# Autodesk Inventor assembly: PIHTI-for-Boron_2026_non-rotating
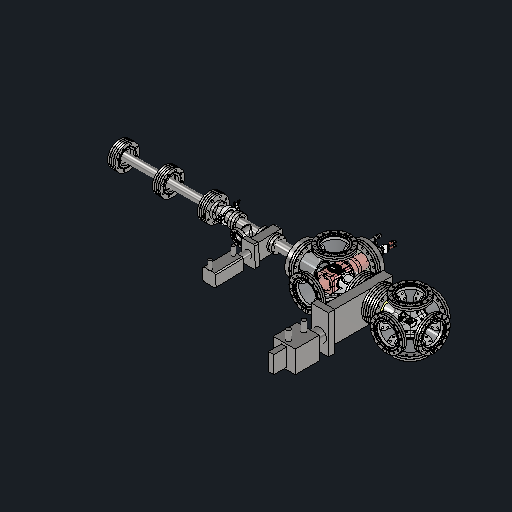
[picture p0: Inventor's stored thumbnail of the model, 512x512]
Saved by Autodesk Inventor 2027.1 (Build 311270010, 270A)
## iProperties
Created: 2024-05-09
Part Number: PIHTI-for-Boron_2026_non-rotating
Document SubType Name: Assembly
Designer: kuzmin
Mass: 19614.5 g
Surface Area: 13609.5 cm^2
Volume: 3689.47 cm^3
Density: 5.31636 g/cm^3
Author: kuzmin
## Documents named in this file (25)
- C:\Users\queezz\Dropbox\Drawings\pihti-cad\Plasma Vessel_2026\PIHTI-for-Boron_2026_non-rotating.iam
- C:\Users\queezz\Dropbox\Drawings\pihti-cad\Plasma Vessel\Plasma-vacuum-cross\Plasma-vacuum-vessel-152IC-cross.iam
- C:\Users\queezz\Dropbox\Drawings\pihti-cad\Plasma Vessel\Plasma-Box\Plasma-box-hayashi-aka-upgrade.iam
- C:\Users\queezz\Dropbox\Drawings\pihti-cad\ContentCenter\Fastners\M3x8-SHCS.ipt
- C:\Users\queezz\Dropbox\Drawings\pihti-cad\Plasma Vessel\Plasma-Box\probe-gate-with-spindel.iam
- C:\Users\queezz\Dropbox\Drawings\pihti-cad\Plasma Vessel\Cathode-Anode-Flange\cf70_spacer.ipt
- C:\Users\queezz\Dropbox\Drawings\pihti-cad\Plasma Vessel\entrance-mesh-assembly.iam
- C:\Users\queezz\Dropbox\Drawings\pihti-cad\Plasma Vessel\probe-port-mesh-welded.iam
- C:\Users\queezz\Dropbox\Drawings\pihti-cad\ContentCenter\CF-parts\CF70-nipple\CF70-nipple.iam
- C:\Users\queezz\Dropbox\Drawings\pihti-cad\ContentCenter\CF-parts\CF70-gate-valve\Gatevalve_70_pneumatic.iam
- C:\Users\queezz\Dropbox\Drawings\pihti-cad\Plasma Vessel_2026\gate_valve\CF150-gatevalve-assembly.iam
- C:\Users\queezz\Dropbox\Drawings\pihti-cad\Plasma Vessel_2026\Plasma-vacuum-vessel\Plasma-vacuum-vessel-152IC-cross-L205p8.iam
- C:\Users\queezz\Dropbox\Drawings\pihti-cad\ContentCenter\CF-parts\CF-70-Tee.ipt
- C:\Users\queezz\Dropbox\Drawings\pihti-cad\ContentCenter\CF-KF-adapters\ICF70_to_KF40.ipt
- C:\Users\queezz\Dropbox\Drawings\pihti-cad\Plasma Vessel\Cathode-Anode-Flange\Cathode-Anode-70IC-flange-with-feeds.iam
- C:\Users\queezz\Dropbox\Drawings\pihti-cad\Plasma Vessel\Plasma-Flange-2024\cathode-box-on-a-flange.iam
- C:\Users\queezz\Dropbox\Drawings\pihti-cad\BoronProbe_2026\BoronProbe_2026.iam
- C:\Users\queezz\Dropbox\Drawings\pihti-cad\ContentCenter\NW\NW40_viton_centering_ring.ipt
- C:\Users\queezz\Dropbox\Drawings\pihti-cad\ContentCenter\NW\NW40_clamp.ipt
- C:\Users\queezz\Dropbox\Drawings\pihti-cad\Plasma Vessel_2026\contents\CF_152-70_bearing.ipt
- C:\Users\queezz\Dropbox\Drawings\pihti-cad\Plasma Vessel_2026\contents\M4×12-VentedHexBolt.ipt
- C:\Users\queezz\Dropbox\Drawings\pihti-cad\BoronProbe_2026\BoronProbe_2026_non-rotating.iam
- C:\Users\queezz\Dropbox\Drawings\pihti-cad\Plasma Vessel_2026\contents\ICF152_bearing_1.ipt
- C:\Users\queezz\Dropbox\Drawings\pihti-cad\BoronProbe_2026\parts\B_probe_bearing_without_holes.ipt
- C:\Users\queezz\Dropbox\Drawings\pihti-cad\BoronProbe_2026\parts\B_probe_bearing.ipt
## Components (35 placed, 23 different names)
1. Plasma-vacuum-vessel-152IC-cross:1 [sub-assembly] — Mate:1, Flush:1, Flush:2, Rigid:18, Mate:22, Mate:23, Mate:24, Mate:59, Mate:60
2. Plasma-box-hayashi-aka-upgrade:1 [sub-assembly] — Mate:3, Mate:4, Hinge Angle, Mate:13, Mate:17
3. probe-gate-with-spindel:1 [sub-assembly] — Mate:3, Mate:4, Hinge Angle
4. cf70_spacer:1 — Mate:61, Mate:62, Mate:63, Mate:64
5. entrance-mesh-assembly:1 [sub-assembly] — Mate:13, Mate:17, Mate:19
6. probe-port-mesh-welded:1 [sub-assembly] — Mate:19
7. CF_152-70_bearing:1 — Rigid:18, Rigid:21, Mate:95, Mate:96, Mate:97
8. CF70-nipple:1 [sub-assembly] — Rigid:21, Rigid:22
9. Gatevalve_70_pneumatic:1 [sub-assembly] — Rigid:22, Mate:47, Mate:48, Mate:49
10. gate_valve_assembly:1 [sub-assembly] — Mate:22, Mate:23, Mate:24, Mate:45, Mate:46, Mate:83, Mate:84, Angle:2
11. Plasma-vacuum-vessel-152IC-cross-L205p8:1 [sub-assembly] — Mate:45, Mate:46, Mate:94
12. CF-70-Tee:1 — Mate:47, Mate:48, Mate:49, Mate:50, Mate:51, Mate:52
13. ICF70_to_KF40:1 — Mate:50, Mate:51, Mate:52, Mate:67, Mate:68, Mate:70, Mate:71
14. Cathode-Anode-70IC-flange-with-feeds:1 [sub-assembly] — Mate:63, Mate:64
15. cathode-box-on-a-flange:1 [sub-assembly] — Mate:59, Mate:60, Mate:61, Mate:62
16. NW40_viton_centering_ring:1 — Mate:67, Mate:68, Mate:81, Mate:82
17. NW40_clamp:1 — Mate:70, Mate:71
18. M4×12-VentedHexBolt:1 — Mate:100, Mate:101
19. M4×12-VentedHexBolt:2 — Mate:98, Mate:99
20. M4×12-VentedHexBolt:3 — Mate:102, Mate:103
21. BoronProbe_2026_non-rotating:1 [sub-assembly] — Mate:81, Mate:82
22. ICF152_bearing_1:1 — Mate:83, Mate:84, Angle:2, Mate:85, Mate:86, Mate:87, Mate:94
23. B_probe_bearing_without_holes:1 — Mate:85, Mate:86, Mate:87, Mate:88, Mate:89, Mate:90, Mate:91, Mate:92, Mate:93
24. M4×12-VentedHexBolt:4 — Mate:88, Mate:89
25. M4×12-VentedHexBolt:5 — Mate:90, Mate:91
26. M4×12-VentedHexBolt:6 — Mate:92, Mate:93
27. B_probe_bearing:1 — Mate:95, Mate:96, Mate:97, Mate:98, Mate:99, Mate:100, Mate:101, Mate:102, Mate:103
28. SS ISO 4762 M3 x 8:5
29. SS ISO 4762 M3 x 8:6
30. SS ISO 4762 M3 x 8:7
31. SS ISO 4762 M3 x 8:8
32. SS ISO 4762 M3 x 8:1
33. SS ISO 4762 M3 x 8:2
34. SS ISO 4762 M3 x 8:3
35. SS ISO 4762 M3 x 8:4
## Relationships (57: Mate 50, WeldJoint 3, Flush 2, Angle 2)
- Mate:1: Plasma-vacuum-vessel-152IC-cross:1
- Flush:1: Plasma-vacuum-vessel-152IC-cross:1
- Flush:2: Plasma-vacuum-vessel-152IC-cross:1
- Mate:3: Plasma-box-hayashi-aka-upgrade:1 ↔ probe-gate-with-spindel:1
- Mate:4: Plasma-box-hayashi-aka-upgrade:1 ↔ probe-gate-with-spindel:1
- Hinge Angle [Angle] (45 deg): Plasma-box-hayashi-aka-upgrade:1 ↔ probe-gate-with-spindel:1
- Mate:13: Plasma-box-hayashi-aka-upgrade:1 ↔ entrance-mesh-assembly:1
- Mate:17: Plasma-box-hayashi-aka-upgrade:1 ↔ entrance-mesh-assembly:1
- Mate:19: entrance-mesh-assembly:1 ↔ probe-port-mesh-welded:1
- Rigid:18 [WeldJoint]: Plasma-vacuum-vessel-152IC-cross:1 ↔ CF_152-70_bearing:1
- Rigid:21 [WeldJoint]: CF_152-70_bearing:1 ↔ CF70-nipple:1
- Rigid:22 [WeldJoint]: CF70-nipple:1 ↔ Gatevalve_70_pneumatic:1
- Mate:22: Plasma-vacuum-vessel-152IC-cross:1 ↔ gate_valve_assembly:1
- Mate:23: Plasma-vacuum-vessel-152IC-cross:1 ↔ gate_valve_assembly:1
- Mate:24: Plasma-vacuum-vessel-152IC-cross:1 ↔ gate_valve_assembly:1
- Mate:45: gate_valve_assembly:1 ↔ Plasma-vacuum-vessel-152IC-cross-L205p8:1
- Mate:46: gate_valve_assembly:1 ↔ Plasma-vacuum-vessel-152IC-cross-L205p8:1
- Mate:47: Gatevalve_70_pneumatic:1 ↔ CF-70-Tee:1
- Mate:48: Gatevalve_70_pneumatic:1 ↔ CF-70-Tee:1
- Mate:49: Gatevalve_70_pneumatic:1 ↔ CF-70-Tee:1
- Mate:50: CF-70-Tee:1 ↔ ICF70_to_KF40:1
- Mate:51: CF-70-Tee:1 ↔ ICF70_to_KF40:1
- Mate:52: CF-70-Tee:1 ↔ ICF70_to_KF40:1
- Mate:59: Plasma-vacuum-vessel-152IC-cross:1 ↔ cathode-box-on-a-flange:1
- Mate:60: Plasma-vacuum-vessel-152IC-cross:1 ↔ cathode-box-on-a-flange:1
- Mate:61: cf70_spacer:1 ↔ cathode-box-on-a-flange:1
- Mate:62: cf70_spacer:1 ↔ cathode-box-on-a-flange:1
- Mate:63: cf70_spacer:1 ↔ Cathode-Anode-70IC-flange-with-feeds:1
- Mate:64: cf70_spacer:1 ↔ Cathode-Anode-70IC-flange-with-feeds:1
- Mate:67: ICF70_to_KF40:1 ↔ NW40_viton_centering_ring:1
- Mate:68: ICF70_to_KF40:1 ↔ NW40_viton_centering_ring:1
- Mate:70: ICF70_to_KF40:1 ↔ NW40_clamp:1
- Mate:71: ICF70_to_KF40:1 ↔ NW40_clamp:1
- Mate:81: NW40_viton_centering_ring:1 ↔ BoronProbe_2026_non-rotating:1
- Mate:82: NW40_viton_centering_ring:1 ↔ BoronProbe_2026_non-rotating:1
- Mate:83: gate_valve_assembly:1 ↔ ICF152_bearing_1:1
- Mate:84: gate_valve_assembly:1 ↔ ICF152_bearing_1:1
- Angle:2 (0 deg): gate_valve_assembly:1 ↔ ICF152_bearing_1:1
- Mate:85: ICF152_bearing_1:1 ↔ B_probe_bearing_without_holes:1
- Mate:86: ICF152_bearing_1:1 ↔ B_probe_bearing_without_holes:1
- Mate:87: ICF152_bearing_1:1 ↔ B_probe_bearing_without_holes:1
- Mate:88: B_probe_bearing_without_holes:1 ↔ M4×12-VentedHexBolt:4
- Mate:89: B_probe_bearing_without_holes:1 ↔ M4×12-VentedHexBolt:4
- Mate:90: B_probe_bearing_without_holes:1 ↔ M4×12-VentedHexBolt:5
- Mate:91: B_probe_bearing_without_holes:1 ↔ M4×12-VentedHexBolt:5
- Mate:92: B_probe_bearing_without_holes:1 ↔ M4×12-VentedHexBolt:6
- Mate:93: B_probe_bearing_without_holes:1 ↔ M4×12-VentedHexBolt:6
- Mate:94: Plasma-vacuum-vessel-152IC-cross-L205p8:1 ↔ ICF152_bearing_1:1
- Mate:95: CF_152-70_bearing:1 ↔ B_probe_bearing:1
- Mate:96: CF_152-70_bearing:1 ↔ B_probe_bearing:1
- Mate:97: CF_152-70_bearing:1 ↔ B_probe_bearing:1
- Mate:98: M4×12-VentedHexBolt:2 ↔ B_probe_bearing:1
- Mate:99: M4×12-VentedHexBolt:2 ↔ B_probe_bearing:1
- Mate:100: M4×12-VentedHexBolt:1 ↔ B_probe_bearing:1
- Mate:101: M4×12-VentedHexBolt:1 ↔ B_probe_bearing:1
- Mate:102: M4×12-VentedHexBolt:3 ↔ B_probe_bearing:1
- Mate:103: M4×12-VentedHexBolt:3 ↔ B_probe_bearing:1
## Named parameters: ProbePos = 738 mm
